# Autodesk Inventor assembly: T-Motor F1507
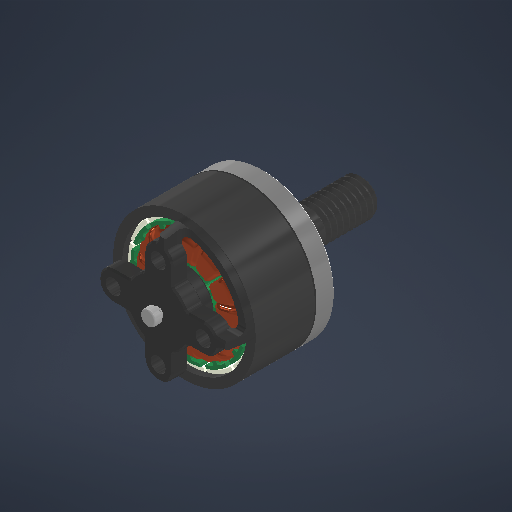
[picture p0: Inventor's stored thumbnail of the model, 512x512]
Saved by Autodesk Inventor 2026.1 (Build 301233020, 233B)
## iProperties
Created: 1601-01-02
Part Number: T-Motor F1507
Document SubType Name: Assembly
Designer: Bahaa
Mass: 18.1842 g
Surface Area: 73.0477 cm^2
Volume: 2.7415 cm^3
Density: 6.63295 g/cm^3
Sending System: SOLIDWORKS 2019
Dibujó: D.Correa
Material: Ver Partes Individuales
Área Sup.: Ver Partes Individuales
last saved by: DanielC
Author: Bahaa
## Documents named in this file (5)
- C:\Users\Bahaa\Nextcloud2\CAD\25-26\V2\Dribbler\Dribbler V2\t-motor-f1507-1.snapshot.1\T-Motor F1507\T-Motor F1507\T-Motor F1507.iam
- C:\Users\Bahaa\Nextcloud2\CAD\25-26\V2\Dribbler\Dribbler V2\t-motor-f1507-1.snapshot.1\T-Motor F1507\T-Motor F1507\Rotor Motor.ipt
- C:\Users\Bahaa\Nextcloud2\CAD\25-26\V2\Dribbler\Dribbler V2\t-motor-f1507-1.snapshot.1\T-Motor F1507\T-Motor F1507\Case Motor.ipt
- C:\Users\Bahaa\Nextcloud2\CAD\25-26\V2\Dribbler\Dribbler V2\t-motor-f1507-1.snapshot.1\T-Motor F1507\T-Motor F1507\Imánes.ipt
- C:\Users\Bahaa\Nextcloud2\CAD\25-26\V2\Dribbler\Dribbler V2\t-motor-f1507-1.snapshot.1\T-Motor F1507\T-Motor F1507\Embobinado.ipt
## Components (4 placed, 4 different names)
1. Rotor Motor-1 — Mate:1, Mate:2
2. Case Motor-1 — Mate:1, Mate:2
3. Imánes-1
4. Embobinado-1
## Relationships (2: Mate 2)
- Mate:1: Rotor Motor-1 ↔ Case Motor-1
- Mate:2: Rotor Motor-1 ↔ Case Motor-1
